# Autodesk Inventor assembly: fullGripperAssembly
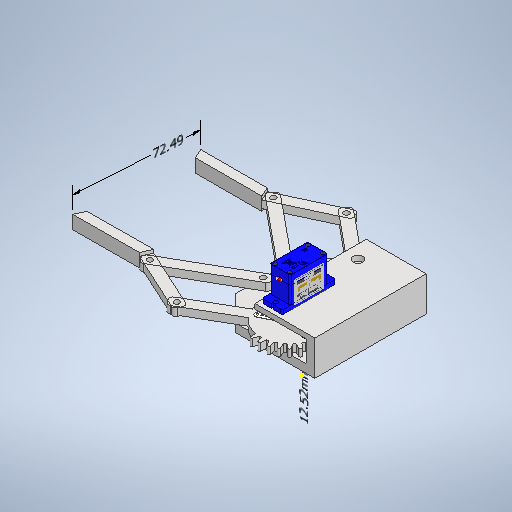
[picture p0: Inventor's stored thumbnail of the model, 512x512]
Saved by Autodesk Inventor 2025.1 (Build 291241020, 241B)
## iProperties
Created: 2025-03-19
Part Number: fullGripperAssembly
Document SubType Name: Assembly
Designer: omiye
Author: omiye
## Documents named in this file (9)
- C:\Projects\Arduino\MazeRobot\models\gripper\fullGripperAssembly.iam
- C:\Projects\Arduino\MazeRobot\models\gripper\base.ipt
- C:\Projects\Arduino\MazeRobot\models\gripper\servoGear.ipt
- C:\Projects\Arduino\MazeRobot\models\gripper\otherGear.ipt
- C:\Projects\Arduino\MazeRobot\models\sg90\sg90body.ipt
- C:\Projects\Arduino\MazeRobot\models\sg90\sg90horn.ipt
- C:\Projects\Arduino\MazeRobot\models\gripper\extension.ipt
- C:\Projects\Arduino\MazeRobot\models\gripper\arm.ipt
- C:\Projects\Arduino\MazeRobot\models\gripper\armMirror.ipt
## Components (9 placed, 8 different names)
1. base:1 — Mate:1, Mate:2, Mate:3, Mate:9, Mate:10, Mate:11, Mate:12, Mate:13, Mate:14, Mate:15
2. sg90body:1 — Mate:1, Mate:2, Mate:3, Mate:4, Mate:5, Mate:7, Mate:9, Mate:10, Mate:11
3. sg90horn:1 — Mate:4, Mate:5, Mate:6, Mate:8
4. servoGear:1 — Mate:6, Mate:7, Mate:8, Flush:1, Mate:18, Flush:5
5. otherGear:1 — Flush:1, Mate:12, Mate:13, Flush:2, Mate:16
6. extension:1 — Flush:3, Mate:15, Mate:19
7. extension:2 — Mate:14, Flush:2, Flush:3, Flush:4, Mate:17
8. arm:1 — Mate:16, Flush:4, Mate:17
9. armMirror:1 — Mate:18, Flush:5, Mate:19
## Relationships (24: Mate 19, Flush 5)
- Mate:1: base:1 ↔ sg90body:1
- Mate:2: base:1 ↔ sg90body:1
- Mate:3: base:1 ↔ sg90body:1
- Mate:4: sg90body:1 ↔ sg90horn:1
- Mate:5: sg90body:1 ↔ sg90horn:1
- Mate:6: sg90horn:1 ↔ servoGear:1
- Mate:7: sg90body:1 ↔ servoGear:1
- Mate:8: sg90horn:1 ↔ servoGear:1
- Mate:9: base:1 ↔ sg90body:1
- Mate:10: base:1 ↔ sg90body:1
- Mate:11: base:1 ↔ sg90body:1
- Flush:1: servoGear:1 ↔ otherGear:1
- Mate:12: base:1 ↔ otherGear:1
- Mate:13: base:1 ↔ otherGear:1
- Mate:14: base:1 ↔ extension:2
- Flush:2: otherGear:1 ↔ extension:2
- Flush:3: extension:1 ↔ extension:2
- Mate:15: base:1 ↔ extension:1
- Mate:16: otherGear:1 ↔ arm:1
- Flush:4: extension:2 ↔ arm:1
- Mate:17: extension:2 ↔ arm:1
- Mate:18: servoGear:1 ↔ armMirror:1
- Flush:5: servoGear:1 ↔ armMirror:1
- Mate:19: extension:1 ↔ armMirror:1
